# Autodesk Inventor assembly: TELJES9
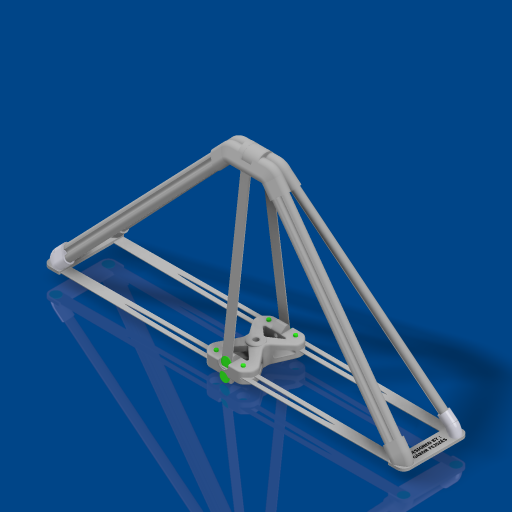
[picture p0: Inventor's stored thumbnail of the model, 512x512]
Saved by Autodesk Inventor 2023 (Build 270158000, 158)
## iProperties
Created: 2022-11-18
Part Number: TELJES9
Document SubType Name: Assembly
Designer: gd1
Author: gd1
## Documents named in this file (3)
- C:\Users\gd1\3D Objects\3D nagyteherbírású híd\Híd\H-d\TELJES9.iam
- C:\Users\gd1\3D Objects\3D nagyteherbírású híd\Híd\H-d\teljes8.iam
- C:\Users\gd1\3D Objects\3D nagyteherbírású híd\Híd\H-d\teljes7.iam
## Components (2 placed, 2 different names)
1. teljes8:1 [sub-assembly] — Rigid:1
2. teljes7:1 [sub-assembly] — Rigid:1
## Relationships (1: WeldJoint 1)
- Rigid:1 [WeldJoint]: teljes8:1 ↔ teljes7:1
